# Autodesk Inventor assembly: Assembly2
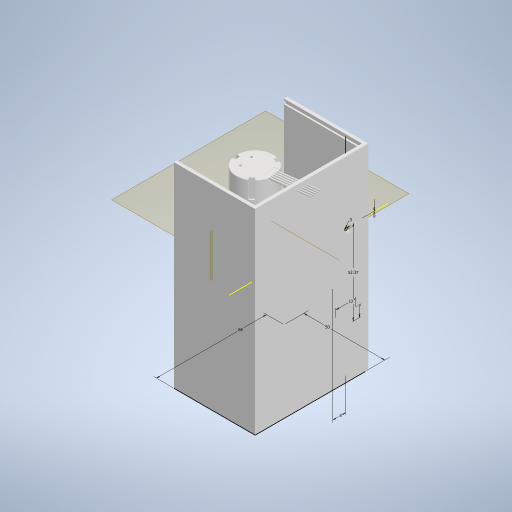
[picture p0: Inventor's stored thumbnail of the model, 512x512]
Saved by Autodesk Inventor 2023 (Build 270158030, 158C)
## iProperties
Created: 2023-03-21
Part Number: Assembly2
Document SubType Name: Assembly
Designer: jxl19
Author: jxl19
## Documents named in this file (8)
- \\icnas3.cc.ic.ac.uk\jxl19\CDPR yr 4\Assembly2.iam
- \\icnas3.cc.ic.ac.uk\jxl19\CDPR yr 4\mar version\spool_3.ipt
- \\icnas3.cc.ic.ac.uk\jxl19\CDPR yr 4\mar version\coupler.ipt
- \\icnas3.cc.ic.ac.uk\jxl19\CDPR yr 4\mar version\encoder_magnet_holder.ipt
- \\icnas3.cc.ic.ac.uk\jxl19\CDPR yr 4\bought components\drawing_16n78.ipt
- \\icnas3.cc.ic.ac.uk\jxl19\CDPR yr 4\bought components\TAL221 500g load cell v1.ipt
- \\icnas3.cc.ic.ac.uk\jxl19\CDPR yr 4\bought components\AEAT-601B Encoder Assembly.ipt
- \\icnas3.cc.ic.ac.uk\jxl19\CDPR yr 4\motor_maincase1.ipt
## Components (7 placed, 7 different names)
1. spool_3:1 — Mate:1
2. coupler:1 — Insert:2, Mate:1
3. encoder_magnet_holder:1 — Mate:2, Mate:3
4. drawing_16n78:1 — Insert:1, Insert:2
5. TAL221 500g load cell v1:1 — Mate:4
6. AEAT-601B Encoder Assembly:1 — Mate:2
7. motor_maincase1:1 — Insert:1, Mate:3, Mate:4
## Relationships (6: Mate 4, Insert 2)
- Insert:1 (3.5 mm): drawing_16n78:1 ↔ motor_maincase1:1
- Insert:2 (-9 mm): coupler:1 ↔ drawing_16n78:1
- Mate:1: spool_3:1 ↔ coupler:1
- Mate:2: encoder_magnet_holder:1 ↔ AEAT-601B Encoder Assembly:1
- Mate:3: encoder_magnet_holder:1 ↔ motor_maincase1:1
- Mate:4: TAL221 500g load cell v1:1 ↔ motor_maincase1:1
